# Autodesk Inventor assembly: 60 Tooth Round Insert
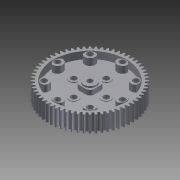
[picture p0: Inventor's stored thumbnail of the model, 180x180]
Saved by Autodesk Inventor 2014 SP1 (Build 180222100, 222)
## iProperties
Created: 2011-05-12
Part Number: 60 Tooth Round Insert
Document SubType Name: Assembly
Designer: Andrew
Author: Andrew
## Documents named in this file (3)
- C:\Users\Ryan\Desktop\sw\lib\Aperture VEX CAD Library\Gears\High Strength Gears\60 Tooth Round Insert.iam
- C:\Users\Ryan\Desktop\sw\lib\Aperture VEX CAD Library\Gears\High Strength Gears\HS-GEAR-60TOOTH.ipt
- C:\Users\Ryan\Desktop\sw\lib\Aperture VEX CAD Library\Gears\High Strength Gears\HS-GEAR-INSERT-PLASTIC.ipt
## Components (3 placed, 2 different names)
1. HS-GEAR-60TOOTH:1 — Mate:5, Mate:6
2. HS-GEAR-INSERT-PLASTIC:1 — Mate:5
3. HS-GEAR-INSERT-PLASTIC:2 — Mate:6
## Relationships (6: Mate 6)
- [Mate]: HS-GEAR-60TOOTH:1 ↔ HS-GEAR-INSERT-PLASTIC:1
- [Mate]: HS-GEAR-60TOOTH:1 ↔ HS-GEAR-INSERT-PLASTIC:1
- [Mate]: HS-GEAR-60TOOTH:1 ↔ HS-GEAR-INSERT-PLASTIC:2
- [Mate]: HS-GEAR-60TOOTH:1 ↔ HS-GEAR-INSERT-PLASTIC:2
- Mate:5: HS-GEAR-60TOOTH:1 ↔ HS-GEAR-INSERT-PLASTIC:1
- Mate:6: HS-GEAR-60TOOTH:1 ↔ HS-GEAR-INSERT-PLASTIC:2
